# Autodesk Inventor assembly: robot
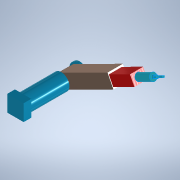
[picture p0: Inventor's stored thumbnail of the model, 180x180]
Saved by Autodesk Inventor 2022 (Build 260153000, 153)
## iProperties
Created: 2022-06-07
Part Number: robot
Document SubType Name: Assembly
Designer: admin
Author: admin
## Documents named in this file (5)
- C:\Users\admin\Dropbox\semestr 4\Modelowanie i sterowanie robotów\laboratoria\projekcik\robocik.iam
- C:\Users\admin\Dropbox\semestr 4\Modelowanie i sterowanie robotów\laboratoria\projekcik\1przegub.ipt
- C:\Users\admin\Dropbox\semestr 4\Modelowanie i sterowanie robotów\laboratoria\projekcik\czesc2.ipt
- C:\Users\admin\Dropbox\semestr 4\Modelowanie i sterowanie robotów\laboratoria\projekcik\czesc3.ipt
- C:\Users\admin\Dropbox\semestr 4\Modelowanie i sterowanie robotów\laboratoria\projekcik\czesc5.ipt
## Components (4 placed, 4 different names)
1. 1przegub:1 — Obrotowe:1
2. czesc2:1 — przesuwne:1, Obrotowe:1
3. czesc3:1 — przesuwne:1, Obrotowe:2
4. czesc5:1 — Obrotowe:2
## Relationships (3: RevoluteJoint 2, TranslationJoint 1)
- przesuwne:1 [TranslationJoint]: czesc2:1 ↔ czesc3:1
- Obrotowe:1 [RevoluteJoint]: 1przegub:1 ↔ czesc2:1
- Obrotowe:2 [RevoluteJoint]: czesc3:1 ↔ czesc5:1
